# Autodesk Inventor assembly: FingerThumb
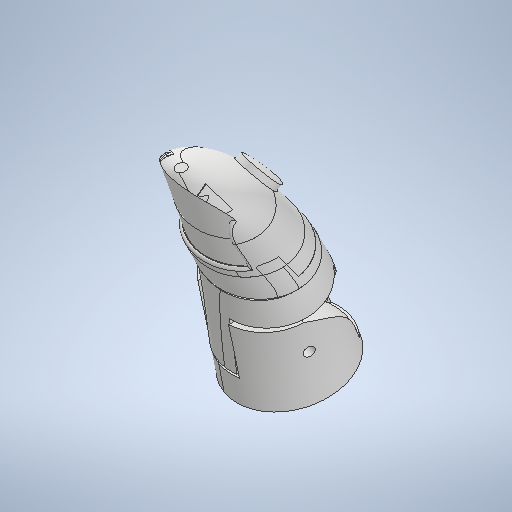
[picture p0: Inventor's stored thumbnail of the model, 512x512]
Saved by Autodesk Inventor 2025.1 (Build 291241000, 241)
## iProperties
Created: 2024-10-03
Part Number: FingerThumb
Document SubType Name: Assembly
Designer: Alexander
Author: Alexander
## Documents named in this file (7)
- D:\Repositorios_Politecnica\Handi-EPN\CAD\Sim Models\FingerThumb.iam
- D:\Repositorios_Politecnica\Handi-EPN\CAD\thumb\DP - D TipTH.ipt
- D:\Repositorios_Politecnica\Handi-EPN\CAD\thumb\DP - D FSR ActuatorTH.ipt
- D:\Repositorios_Politecnica\Handi-EPN\CAD\thumb\DP - D MainTH.ipt
- D:\Repositorios_Politecnica\Handi-EPN\CAD\thumb\DP - D LockTH.ipt
- D:\Repositorios_Politecnica\Handi-EPN\CAD\thumb\DP - P MainTH R.ipt
- D:\Repositorios_Politecnica\Handi-EPN\CAD\thumb\IP - DTH R.ipt
## Components (6 placed, 6 different names)
1. DP - D TipTH:1 — Mate:3, Mate:4
2. DP - D FSR ActuatorTH:1 — Mate:1, Mate:2, Mate:4
3. DP - D MainTH:1 — Mate:1, Mate:2, Mate:3, Mate:5, Flush:1, Flush:2
4. DP - D LockTH:1 — Mate:5, Flush:1, Flush:2, Mate:6, Mate:7
5. DP - P MainTH R:1 — Mate:6, Mate:7, Rotational:1
6. IP - DTH R:1 — Rotational:1
## Relationships (10: Mate 7, Flush 2, RevoluteJoint 1)
- Mate:1: DP - D FSR ActuatorTH:1 ↔ DP - D MainTH:1
- Mate:2: DP - D FSR ActuatorTH:1 ↔ DP - D MainTH:1
- Mate:3: DP - D TipTH:1 ↔ DP - D MainTH:1
- Mate:4: DP - D TipTH:1 ↔ DP - D FSR ActuatorTH:1
- Mate:5: DP - D MainTH:1 ↔ DP - D LockTH:1
- Flush:1: DP - D MainTH:1 ↔ DP - D LockTH:1
- Flush:2: DP - D MainTH:1 ↔ DP - D LockTH:1
- Mate:6: DP - D LockTH:1 ↔ DP - P MainTH R:1
- Mate:7: DP - D LockTH:1 ↔ DP - P MainTH R:1
- Rotational:1 [RevoluteJoint] (-2 mm): DP - P MainTH R:1 ↔ IP - DTH R:1
